# Autodesk Inventor assembly: pulsador
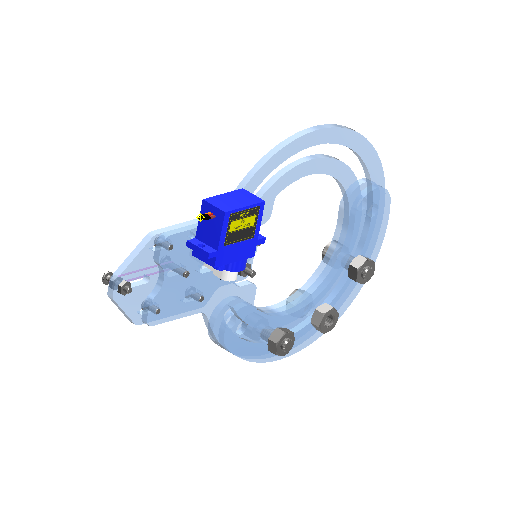
[picture p0: Inventor's stored thumbnail of the model, 512x512]
Saved by Autodesk Inventor 2022 (Build 260153000, 153)
## iProperties
Created: 2022-11-16
Part Number: pulsador
Document SubType Name: Assembly
Designer: ferna
Author: ferna
## Documents named in this file (12)
- C:\Users\ferna\Documents\Bocas\Prototipo_09\New folder\pulsador - 7.iam
- C:\Users\ferna\Documents\Bocas\Prototipo_09\New folder\pulsador_monta_riel.ipt
- C:\Users\ferna\Documents\Bocas\Prototipo_09\New folder\pulsador_monta_servo.ipt
- C:\Users\ferna\Documents\Bocas\Prototipo_09\New folder\pulsador_presion.ipt
- C:\Users\ferna\Documents\Bocas\Prototipo_09\New folder\pulsador_punta.ipt
- C:\Users\ferna\Documents\Bocas\Prototipo_09\New folder\servo.ipt
- C:\Users\ferna\Documents\Inventor\Content Center Files\R2022\en-US\Screw GB_T 70.2\Screw GB_T 70.2 M3 X 6.ipt
- C:\Users\ferna\Documents\Inventor\Content Center Files\R2022\en-US\Screw GB_T 70.2\Screw GB_T 70.2 M3 X 12.ipt
- C:\Users\ferna\Documents\Inventor\Content Center Files\R2022\en-US\AS 1474(1)\AS 1474 - M3(1).ipt
- C:\Users\ferna\Documents\Bocas\Prototipo_09\New folder\elastico.ipt
- C:\Users\ferna\Documents\Inventor\Content Center Files\R2022\en-US\AS 1112 (2)\AS 1112 - M6  Type 5.ipt
- C:\Users\ferna\Documents\Inventor\Content Center Files\R2022\en-US\CSN 02 1143  B\CSN 02 1143 - M6 x 1 x 16(2).ipt
## Components (25 placed, 11 different names)
1. pulsador_monta_riel:1 — Mate:1, Flush:1, Flush:2, Mate:5, Mate:6, Mate:7, Mate:10, Mate:11, Tangent:1, Mate:12, Mate:13, Mate:14, Mate:15, Mate:20, Angle:2
2. pulsador_monta_servo:1 — Mate:1, Flush:1, Mate:2, Mate:3, Mate:4, Flush:2, Angle:1, Mate:16, Mate:17, Mate:18, Mate:19, Mate:22, Mate:23, Mate:26, Mate:27, Mate:28, Mate:29, Mate:34, Mate:35, Mate:38
3. pulsador_presion:1 — Mate:6, Mate:7, Mate:8, Mate:9, Mate:39, Mate:40, Mate:43, Mate:47, Mate:48, Mate:49
4. pulsador_punta:1 — Mate:2, Mate:3, Mate:4, Mate:30, Mate:31
5. pulsador_presion:2 — Mate:5, Mate:8, Mate:9, Angle:1, Mate:44, Mate:45, Mate:46, Mate:50
6. servo:1 — Mate:10, Mate:11, Tangent:1
7. Screw GB/T 70.2 M3 X 6:1 — Mate:12, Mate:19
8. Screw GB/T 70.2 M3 X 6:2 — Mate:13, Mate:16
9. Screw GB/T 70.2 M3 X 6:3 — Mate:14, Mate:18
10. Screw GB/T 70.2 M3 X 6:4 — Mate:15, Mate:17
11. Screw GB/T 70.2 M3 X 12:1 — Mate:20, Mate:23
12. Screw GB/T 70.2 M3 X 12:2 — Mate:22, Mate:24, Mate:25, Mate:36, Mate:38
13. AS 1474 - Metric M3:1 — Mate:24, Mate:26, Mate:37
14. AS 1474 - Metric M3:2 — Mate:25, Mate:27
15. AS 1474 - Metric M3:3 — Mate:33, Mate:34
16. AS 1474 - Metric M3:4 — Mate:32, Mate:35
17. Screw GB/T 70.2 M3 X 12:3 — Mate:28, Mate:31, Mate:32
18. Screw GB/T 70.2 M3 X 12:4 — Mate:29, Mate:30, Mate:33
19. elastico:1 — Mate:36, Angle:2, Mate:37
20. AS 1112 (2) - Metric M6  Type 5:1 — Mate:41, Mate:47
21. AS 1112 (2) - Metric M6  Type 5:2 — Mate:43, Mate:48
22. AS 1112 (2) - Metric M6  Type 5:3 — Mate:42, Mate:49
23. AS 1112 (2) - Metric M6  Type 5:4 — Mate:46, Mate:50
24. CSN 02 1143 B M6 x 16:1 — Mate:39, Mate:41, Mate:45
25. CSN 02 1143 B M6 x 16:2 — Mate:40, Mate:42, Mate:44
## Relationships (54: Mate 49, Flush 2, Angle 2, Tangent 1)
- Mate:1: pulsador_monta_riel:1 ↔ pulsador_monta_servo:1
- Flush:1: pulsador_monta_riel:1 ↔ pulsador_monta_servo:1
- Mate:2: pulsador_monta_servo:1 ↔ pulsador_punta:1
- Mate:3: pulsador_monta_servo:1 ↔ pulsador_punta:1
- Mate:4: pulsador_monta_servo:1 ↔ pulsador_punta:1
- Flush:2 (20 mm): pulsador_monta_riel:1 ↔ pulsador_monta_servo:1
- Mate:5: pulsador_monta_riel:1 ↔ pulsador_presion:2
- Mate:6: pulsador_monta_riel:1 ↔ pulsador_presion:1
- Mate:7: pulsador_monta_riel:1 ↔ pulsador_presion:1
- Mate:8: pulsador_presion:1 ↔ pulsador_presion:2
- Mate:9: pulsador_presion:1 ↔ pulsador_presion:2
- Angle:1 (150 deg): pulsador_monta_servo:1 ↔ pulsador_presion:2
- Mate:10: pulsador_monta_riel:1 ↔ servo:1
- Mate:11 (-0.5 mm): pulsador_monta_riel:1 ↔ servo:1
- Tangent:1 (-0.18 mm): pulsador_monta_riel:1 ↔ servo:1
- Mate:12: pulsador_monta_riel:1 ↔ Screw GB/T 70.2 M3 X 6:1
- Mate:13: pulsador_monta_riel:1 ↔ Screw GB/T 70.2 M3 X 6:2
- Mate:14: pulsador_monta_riel:1 ↔ Screw GB/T 70.2 M3 X 6:3
- Mate:15: pulsador_monta_riel:1 ↔ Screw GB/T 70.2 M3 X 6:4
- Mate:16: pulsador_monta_servo:1 ↔ Screw GB/T 70.2 M3 X 6:2
- Mate:17: pulsador_monta_servo:1 ↔ Screw GB/T 70.2 M3 X 6:4
- Mate:18: pulsador_monta_servo:1 ↔ Screw GB/T 70.2 M3 X 6:3
- Mate:19: pulsador_monta_servo:1 ↔ Screw GB/T 70.2 M3 X 6:1
- Mate:20: pulsador_monta_riel:1 ↔ Screw GB/T 70.2 M3 X 12:1
- Mate:22 (5 mm): pulsador_monta_servo:1 ↔ Screw GB/T 70.2 M3 X 12:2
- Mate:23 (5 mm): pulsador_monta_servo:1 ↔ Screw GB/T 70.2 M3 X 12:1
- Mate:24: Screw GB/T 70.2 M3 X 12:2 ↔ AS 1474 - Metric M3:1
- Mate:25: Screw GB/T 70.2 M3 X 12:2 ↔ AS 1474 - Metric M3:2
- Mate:26: pulsador_monta_servo:1 ↔ AS 1474 - Metric M3:1
- Mate:27: pulsador_monta_servo:1 ↔ AS 1474 - Metric M3:2
- Mate:28: pulsador_monta_servo:1 ↔ Screw GB/T 70.2 M3 X 12:3
- Mate:29: pulsador_monta_servo:1 ↔ Screw GB/T 70.2 M3 X 12:4
- Mate:30: pulsador_punta:1 ↔ Screw GB/T 70.2 M3 X 12:4
- Mate:31: pulsador_punta:1 ↔ Screw GB/T 70.2 M3 X 12:3
- Mate:32: AS 1474 - Metric M3:4 ↔ Screw GB/T 70.2 M3 X 12:3
- Mate:33: AS 1474 - Metric M3:3 ↔ Screw GB/T 70.2 M3 X 12:4
- Mate:34: pulsador_monta_servo:1 ↔ AS 1474 - Metric M3:3
- Mate:35: pulsador_monta_servo:1 ↔ AS 1474 - Metric M3:4
- Mate:36: Screw GB/T 70.2 M3 X 12:2 ↔ elastico:1
- Angle:2 (0 deg): pulsador_monta_riel:1 ↔ elastico:1
- Mate:37: AS 1474 - Metric M3:1 ↔ elastico:1
- Mate:38: pulsador_monta_servo:1 ↔ Screw GB/T 70.2 M3 X 12:2
- Mate:39: pulsador_presion:1 ↔ CSN 02 1143 B M6 x 16:1
- Mate:40: pulsador_presion:1 ↔ CSN 02 1143 B M6 x 16:2
- Mate:41: AS 1112 (2) - Metric M6  Type 5:1 ↔ CSN 02 1143 B M6 x 16:1
- Mate:42: AS 1112 (2) - Metric M6  Type 5:3 ↔ CSN 02 1143 B M6 x 16:2
- Mate:43: pulsador_presion:1 ↔ AS 1112 (2) - Metric M6  Type 5:2
- Mate:44: pulsador_presion:2 ↔ CSN 02 1143 B M6 x 16:2
- Mate:45: pulsador_presion:2 ↔ CSN 02 1143 B M6 x 16:1
- Mate:46: pulsador_presion:2 ↔ AS 1112 (2) - Metric M6  Type 5:4
- Mate:47: pulsador_presion:1 ↔ AS 1112 (2) - Metric M6  Type 5:1
- Mate:48: pulsador_presion:1 ↔ AS 1112 (2) - Metric M6  Type 5:2
- Mate:49: pulsador_presion:1 ↔ AS 1112 (2) - Metric M6  Type 5:3
- Mate:50: pulsador_presion:2 ↔ AS 1112 (2) - Metric M6  Type 5:4
